# Autodesk Inventor assembly: Gripper
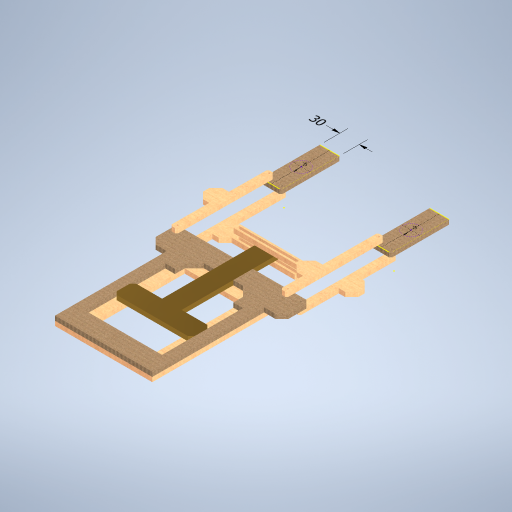
[picture p0: Inventor's stored thumbnail of the model, 512x512]
Saved by Autodesk Inventor 2023.1 (Build 271208000, 208)
## iProperties
Created: 2022-10-28
Part Number: Gripper
Document SubType Name: Assembly
Designer: Daniel Peña
Author: Daniel Peña
## Documents named in this file (7)
- E:\Daniel DiscoA\Documents\UNAL\ProyectoRobotica\CAD\Gripper.iam
- E:\Daniel DiscoA\Documents\UNAL\ProyectoRobotica\CAD\Base.ipt
- E:\Daniel DiscoA\Documents\UNAL\ProyectoRobotica\CAD\Marco.ipt
- E:\Daniel DiscoA\Documents\UNAL\ProyectoRobotica\CAD\Piston.ipt
- E:\Daniel DiscoA\Documents\UNAL\ProyectoRobotica\CAD\Dedo.ipt
- E:\Daniel DiscoA\Documents\UNAL\ProyectoRobotica\CAD\Lever.ipt
- E:\Daniel DiscoA\Documents\UNAL\ProyectoRobotica\CAD\tLever.ipt
## Components (10 placed, 6 different names)
1. Base:1 — Flush:1, Mate:2
2. Marco:1 — Flush:1, Flush:4, Mate:1, Rotational:1, Rotational:7, Mate:3, Mate:4, Rotational:11, Rotational:12
3. Piston:1 — Mate:2, Mate:3, Mate:4
4. Base:2 — Flush:4, Mate:1
5. Dedo:1 — Rotational:2, Rotational:14
6. Dedo:2 — Rotational:10, Rotational:13
7. Lever:1 — Rotational:1, Rotational:2
8. Lever:2 — Rotational:7, Rotational:10
9. tLever:1 — Rotational:12, Rotational:14
10. tLever:2 — Rotational:11, Rotational:13
## Relationships (14: RevoluteJoint 8, Mate 4, Flush 2)
- Flush:1: Base:1 ↔ Marco:1
- Flush:4: Marco:1 ↔ Base:2
- Mate:1: Marco:1 ↔ Base:2
- Rotational:1 [RevoluteJoint]: Marco:1 ↔ Lever:1
- Rotational:2 [RevoluteJoint]: Dedo:1 ↔ Lever:1
- Rotational:7 [RevoluteJoint]: Marco:1 ↔ Lever:2
- Rotational:10 [RevoluteJoint]: Dedo:2 ↔ Lever:2
- Mate:2: Base:1 ↔ Piston:1
- Mate:3: Marco:1 ↔ Piston:1
- Mate:4: Marco:1 ↔ Piston:1
- Rotational:11 [RevoluteJoint]: Marco:1 ↔ tLever:2
- Rotational:12 [RevoluteJoint]: Marco:1 ↔ tLever:1
- Rotational:13 [RevoluteJoint]: Dedo:2 ↔ tLever:2
- Rotational:14 [RevoluteJoint]: Dedo:1 ↔ tLever:1
## Named parameters: hMDF = 7 mm
